# Autodesk Inventor assembly: claw_dynamic_gripper_assembly
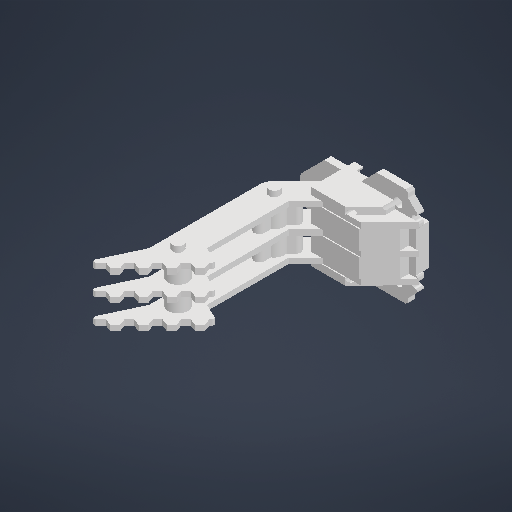
[picture p0: Inventor's stored thumbnail of the model, 512x512]
Saved by Autodesk Inventor 2026 (Build 300175000, 175)
## iProperties
Created: 2025-03-27
Part Number: claw_dynamic_gripper_assembly
Document SubType Name: Assembly
Designer: paris
Author: paris
## Documents named in this file (6)
- C:\Users\paris\OneDrive\Desktop\3d models\claw_dynamic_gripper_assembly.iam
- C:\Users\paris\OneDrive\Desktop\3d models\claw_dynamic_gripper.ipt
- C:\Users\paris\OneDrive\Desktop\3d models\claw_dynamic_mount.ipt
- C:\Users\paris\OneDrive\Desktop\3d models\claw_connecting_rod.ipt
- C:\Users\paris\OneDrive\Desktop\3d models\claw_spacer.ipt
- C:\Users\paris\OneDrive\Desktop\3d models\claw_joined_spacer.ipt
## Components (10 placed, 5 different names)
1. claw_dynamic_gripper:1 — Mate:1, Mate:2, Mate:7, Mate:8, Flush:1, Flush:2, Mate:13, Mate:14
2. claw_dynamic_mount:1 — Mate:1, Mate:2, Mate:3, Mate:4, Mate:5, Mate:6
3. claw_dynamic_gripper:2 — Mate:3, Mate:5, Mate:15, Mate:16, Angle:2, Mate:17
4. claw_dynamic_gripper:3 — Mate:4, Mate:6, Angle:1, Mate:18
5. claw_connecting_rod:1 — Mate:7, Flush:1, Mate:9, Mate:10, Mate:17, Mate:18
6. claw_connecting_rod:2 — Mate:8, Flush:2, Mate:11, Mate:12
7. claw_spacer:1 — Mate:11, Mate:13
8. claw_spacer:2 — Mate:12, Mate:16
9. claw_joined_spacer:1 — Mate:10, Mate:14, Angle:2
10. claw_joined_spacer:2 — Mate:9, Mate:15, Angle:1
## Relationships (22: Mate 18, Flush 2, Angle 2)
- Mate:1: claw_dynamic_gripper:1 ↔ claw_dynamic_mount:1
- Mate:2: claw_dynamic_gripper:1 ↔ claw_dynamic_mount:1
- Mate:3: claw_dynamic_mount:1 ↔ claw_dynamic_gripper:2
- Mate:4: claw_dynamic_mount:1 ↔ claw_dynamic_gripper:3
- Mate:5: claw_dynamic_mount:1 ↔ claw_dynamic_gripper:2
- Mate:6: claw_dynamic_mount:1 ↔ claw_dynamic_gripper:3
- Mate:7: claw_dynamic_gripper:1 ↔ claw_connecting_rod:1
- Mate:8: claw_dynamic_gripper:1 ↔ claw_connecting_rod:2
- Flush:1 (-2 mm): claw_dynamic_gripper:1 ↔ claw_connecting_rod:1
- Flush:2 (-2 mm): claw_dynamic_gripper:1 ↔ claw_connecting_rod:2
- Mate:9: claw_connecting_rod:1 ↔ claw_joined_spacer:2
- Mate:10: claw_connecting_rod:1 ↔ claw_joined_spacer:1
- Mate:11: claw_connecting_rod:2 ↔ claw_spacer:1
- Mate:12: claw_connecting_rod:2 ↔ claw_spacer:2
- Mate:13: claw_dynamic_gripper:1 ↔ claw_spacer:1
- Mate:14: claw_dynamic_gripper:1 ↔ claw_joined_spacer:1
- Mate:15: claw_dynamic_gripper:2 ↔ claw_joined_spacer:2
- Mate:16: claw_dynamic_gripper:2 ↔ claw_spacer:2
- Angle:1 (0 deg): claw_dynamic_gripper:3 ↔ claw_joined_spacer:2
- Angle:2 (0 deg): claw_dynamic_gripper:2 ↔ claw_joined_spacer:1
- Mate:17: claw_dynamic_gripper:2 ↔ claw_connecting_rod:1
- Mate:18: claw_dynamic_gripper:3 ↔ claw_connecting_rod:1
